# Autodesk Inventor assembly: boardroom table
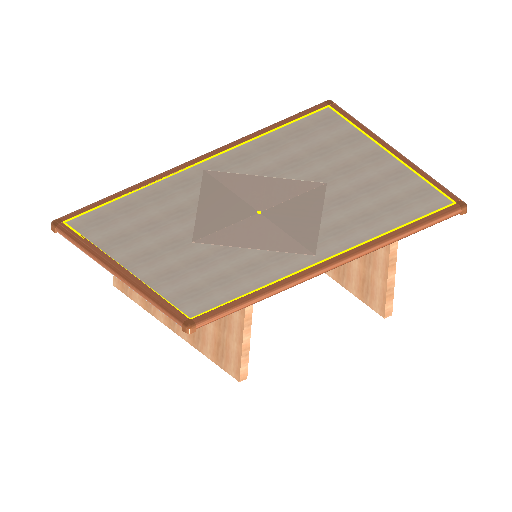
[picture p0: Inventor's stored thumbnail of the model, 512x512]
Saved by Autodesk Inventor 2025 (Build 290162000, 162)
## iProperties
Created: 2024-09-12
Part Number: boardroom table
Document SubType Name: Assembly
Designer: teiko
Author: teiko
## Documents named in this file (3)
- C:\Users\teiko\OneDrive\Documents\Inventor\boardroom\assembly\boardroom table.iam
- C:\Users\teiko\OneDrive\Documents\Inventor\boardroom\table base\assembly\table base assembly.iam
- C:\Users\teiko\OneDrive\Documents\Inventor\boardroom\table top\assembly\table top assembly.iam
## Components (2 placed, 2 different names)
1. table base assembly:1 [sub-assembly] — Mate:1, Mate:2, Mate:3
2. table top assembly:1 [sub-assembly] — Mate:1, Mate:2, Mate:3
## Relationships (3: Mate 3)
- Mate:1: table base assembly:1 ↔ table top assembly:1
- Mate:2: table base assembly:1 ↔ table top assembly:1
- Mate:3: table base assembly:1 ↔ table top assembly:1
